# Autodesk Inventor assembly: expoassemble
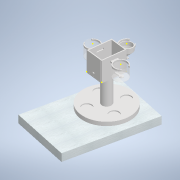
[picture p0: Inventor's stored thumbnail of the model, 180x180]
Saved by Autodesk Inventor 2020 (Build 240168000, 168)
## iProperties
Created: 2020-02-18
Part Number: expoassemble
Document SubType Name: Assembly
Designer: Aryan
Author: Aryan
## Documents named in this file (11)
- C:\Users\Aryan\Documents\expoassemble.iam
- C:\Users\Aryan\Documents\expo2.ipt
- C:\Users\Aryan\Documents\expo3.ipt
- C:\Users\Aryan\Documents\expo4.ipt
- C:\Users\Aryan\Documents\expo5.ipt
- C:\Users\Aryan\Documents\expo7.ipt
- C:\Users\Aryan\Documents\Assembly1.iam
- C:\Users\Aryan\Documents\expo8.ipt
- C:\Users\Aryan\Documents\seeder.ipt
- C:\Users\Aryan\Documents\expo13.ipt
- C:\Users\Aryan\Documents\seddd.ipt
## Components (16 placed, 10 different names)
1. expo2:1 — Mate:1, Mate:2, Flush:1, Mate:3, Mate:4, Flush:2, Mate:5, Mate:6, Mate:7, Mate:8, Flush:3, Flush:4, Mate:26, Mate:27
2. expo3:1 — Mate:1, Mate:2, Flush:1, Rotation:1, Rotation:2, Mate:21, Mate:22, Mate:23
3. expo3:2 — Mate:3, Mate:4, Flush:2, Mate:18, Mate:19, Mate:20
4. expo4:1 — Mate:7, Mate:8, Flush:3
5. expo4:2 — Mate:5, Mate:6, Flush:4, Mate:24, Mate:28
6. expo5:3 — Mate:18, Mate:19, Mate:20, Insert:1
7. expo5:4 — Rotation:1, Rotation:2, Mate:21, Mate:22, Mate:23, Mate:25, Insert:3
8. expo5:5 — Mate:24, Mate:28, Mate:29
9. expo7:1 — Mate:25, Insert:3
10. expo7:2 — Insert:1
11. Assembly1:1 [sub-assembly] — Mate:26, Mate:27, Insert:4
12. expo8:1 — Insert:4
13. seeder:1 — Mate:29
14. expo13:1
15. expo13:2
16. seddd:1
## Relationships (29: Mate 20, Flush 4, Insert 3, RelateRotation 2)
- Mate:1: expo2:1 ↔ expo3:1
- Mate:2: expo2:1 ↔ expo3:1
- Flush:1: expo2:1 ↔ expo3:1
- Mate:3: expo2:1 ↔ expo3:2
- Mate:4: expo2:1 ↔ expo3:2
- Flush:2: expo2:1 ↔ expo3:2
- Mate:5: expo2:1 ↔ expo4:2
- Mate:6: expo2:1 ↔ expo4:2
- Mate:7: expo2:1 ↔ expo4:1
- Mate:8: expo2:1 ↔ expo4:1
- Flush:3: expo2:1 ↔ expo4:1
- Flush:4: expo2:1 ↔ expo4:2
- Mate:18: expo3:2 ↔ expo5:3
- Mate:19: expo3:2 ↔ expo5:3
- Mate:20: expo3:2 ↔ expo5:3
- Rotation:1 [RelateRotation] (1 ul): expo3:1 ↔ expo5:4
- Rotation:2 [RelateRotation] (12 ul): expo3:1 ↔ expo5:4
- Mate:21: expo3:1 ↔ expo5:4
- Mate:22: expo3:1 ↔ expo5:4
- Mate:23: expo3:1 ↔ expo5:4
- Mate:24: expo4:2 ↔ expo5:5
- Mate:25: expo5:4 ↔ expo7:1
- Insert:1: expo5:3 ↔ expo7:2
- Mate:26: expo2:1 ↔ Assembly1:1
- Mate:27: expo2:1 ↔ Assembly1:1
- Insert:3: expo5:4 ↔ expo7:1
- Mate:28: expo4:2 ↔ expo5:5
- Insert:4: Assembly1:1 ↔ expo8:1
- Mate:29: expo5:5 ↔ seeder:1
